# Autodesk Inventor assembly: Lightsaber Assembly 4
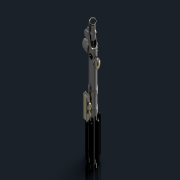
[picture p0: Inventor's stored thumbnail of the model, 180x180]
Saved by Autodesk Inventor 2021 (Build 250183000, 183)
## iProperties
Created: 2021-01-12
Part Number: Lightsaber Assembly 4
Document SubType Name: Assembly
Designer: Alex
Author: Alex
## Documents named in this file (13)
- D:\Documents (HDD)\lightsaber\Lightsaber Assembly 4.iam
- D:\Documents (HDD)\lightsaber\Grip.ipt
- D:\Documents (HDD)\lightsaber\Grip Base.ipt
- D:\Documents (HDD)\lightsaber\pin.ipt
- D:\Documents (HDD)\lightsaber\Middle handle.ipt
- D:\Documents (HDD)\lightsaber\top.ipt
- D:\Documents (HDD)\lightsaber\Clip.ipt
- D:\Documents (HDD)\lightsaber\Pin2.ipt
- D:\Documents (HDD)\lightsaber\Button1.ipt
- D:\Documents (HDD)\lightsaber\emitter.ipt
- D:\Documents (HDD)\lightsaber\Button.ipt
- D:\Documents (HDD)\lightsaber\Switch.ipt
- D:\Documents (HDD)\lightsaber\button 3.ipt
## Components (31 placed, 12 different names)
1. Grip:1 — Mate:1, Mate:2, Mate:49
2. Grip Base:1 — Mate:1, Mate:2, Mate:3, Mate:4, Mate:5, Mate:6, Mate:7, Mate:8, Mate:11, Mate:12, Mate:13, Mate:14, Insert:1, Insert:2, Insert:3, Insert:4, Insert:5, Insert:6, Insert:7, Insert:8, Insert:9, Insert:10, Insert:11, Insert:12, Mate:15, Mate:16, Mate:17
3. Grip:2 — Mate:3, Mate:4, Mate:45
4. Grip:3 — Mate:5, Mate:6, Mate:50
5. Grip:4 — Mate:7, Mate:8, Mate:48
6. Grip:5 — Mate:11, Mate:12, Mate:47
7. Grip:6 — Mate:13, Mate:14, Mate:46
8. pin:1 — Insert:10, Mate:46
9. pin:2 — Insert:9
10. pin:3 — Insert:11
11. pin:4 — Insert:12, Mate:50
12. pin:5 — Insert:7, Mate:47
13. pin:6 — Insert:8
14. pin:7 — Insert:5, Mate:48
15. pin:8 — Insert:6
16. pin:9 — Insert:2, Mate:49
17. pin:10 — Insert:4
18. pin:11 — Insert:1, Mate:45
19. pin:12 — Insert:3
20. Middle handle:1 — Mate:15, Mate:16, Mate:17, Mate:18, Mate:19, Mate:20, Mate:36, Mate:37, Mate:38, Angle:7, Flush:1
21. top:1 — Mate:18, Mate:19, Mate:20, Mate:22, Mate:23, Mate:24, Mate:25, Mate:26, Mate:27, Mate:28, Mate:29, Mate:30, Mate:31, Angle:1, Angle:2, Angle:3, Angle:4, Mate:32, Mate:33, Angle:5, Mate:34, Mate:35, Angle:6, Mate:42, Mate:43, Mate:44
22. Clip:1 — Mate:22, Mate:23
23. Pin2:1 — Mate:24, Mate:25, Angle:4
24. Pin2:2 — Mate:26, Mate:27, Angle:3
25. Pin2:3 — Mate:28, Mate:29, Angle:2
26. Pin2:4 — Mate:30, Mate:31, Angle:1
27. Button1:1 — Mate:32, Mate:33, Angle:5
28. emitter:1 — Mate:34, Mate:35, Angle:6
29. Button:1 — Mate:36, Mate:37, Mate:38, Angle:7, Flush:1, Angle:8, Mate:39, Mate:40, Mate:41
30. Switch:1 — Angle:8, Mate:39, Mate:40, Mate:41
31. button 3:1 — Mate:42, Mate:43, Mate:44
## Relationships (68: Mate 47, Insert 12, Angle 8, Flush 1)
- Mate:1: Grip:1 ↔ Grip Base:1
- Mate:2: Grip:1 ↔ Grip Base:1
- Mate:3: Grip Base:1 ↔ Grip:2
- Mate:4: Grip Base:1 ↔ Grip:2
- Mate:5: Grip Base:1 ↔ Grip:3
- Mate:6: Grip Base:1 ↔ Grip:3
- Mate:7: Grip Base:1 ↔ Grip:4
- Mate:8: Grip Base:1 ↔ Grip:4
- Mate:11: Grip Base:1 ↔ Grip:5
- Mate:12: Grip Base:1 ↔ Grip:5
- Mate:13: Grip Base:1 ↔ Grip:6
- Mate:14: Grip Base:1 ↔ Grip:6
- Insert:1: Grip Base:1 ↔ pin:11
- Insert:2: Grip Base:1 ↔ pin:9
- Insert:3: Grip Base:1 ↔ pin:12
- Insert:4: Grip Base:1 ↔ pin:10
- Insert:5: Grip Base:1 ↔ pin:7
- Insert:6: Grip Base:1 ↔ pin:8
- Insert:7: Grip Base:1 ↔ pin:5
- Insert:8: Grip Base:1 ↔ pin:6
- Insert:9: Grip Base:1 ↔ pin:2
- Insert:10: Grip Base:1 ↔ pin:1
- Insert:11: Grip Base:1 ↔ pin:3
- Insert:12: Grip Base:1 ↔ pin:4
- Mate:15: Grip Base:1 ↔ Middle handle:1
- Mate:16: Grip Base:1 ↔ Middle handle:1
- Mate:17: Grip Base:1 ↔ Middle handle:1
- Mate:18: Middle handle:1 ↔ top:1
- Mate:19: Middle handle:1 ↔ top:1
- Mate:20: Middle handle:1 ↔ top:1
- Mate:22: top:1 ↔ Clip:1
- Mate:23: top:1 ↔ Clip:1
- Mate:24: top:1 ↔ Pin2:1
- Mate:25: top:1 ↔ Pin2:1
- Mate:26: top:1 ↔ Pin2:2
- Mate:27: top:1 ↔ Pin2:2
- Mate:28: top:1 ↔ Pin2:3
- Mate:29: top:1 ↔ Pin2:3
- Mate:30: top:1 ↔ Pin2:4
- Mate:31: top:1 ↔ Pin2:4
- Angle:1 (180 deg): top:1 ↔ Pin2:4
- Angle:2 (0 deg): top:1 ↔ Pin2:3
- Angle:3 (0 deg): top:1 ↔ Pin2:2
- Angle:4 (0 deg): top:1 ↔ Pin2:1
- Mate:32: top:1 ↔ Button1:1
- Mate:33: top:1 ↔ Button1:1
- Angle:5 (0 deg): top:1 ↔ Button1:1
- Mate:34: top:1 ↔ emitter:1
- Mate:35: top:1 ↔ emitter:1
- Angle:6 (0 deg): top:1 ↔ emitter:1
- Mate:36: Middle handle:1 ↔ Button:1
- Mate:37: Middle handle:1 ↔ Button:1
- Mate:38: Middle handle:1 ↔ Button:1
- Angle:7 (0 deg): Middle handle:1 ↔ Button:1
- Flush:1: Middle handle:1 ↔ Button:1
- Angle:8 (0 deg): Button:1 ↔ Switch:1
- Mate:39: Button:1 ↔ Switch:1
- Mate:40 (1 mm): Button:1 ↔ Switch:1
- Mate:41 (1 mm): Button:1 ↔ Switch:1
- Mate:42: top:1 ↔ button 3:1
- Mate:43: top:1 ↔ button 3:1
- Mate:44: top:1 ↔ button 3:1
- Mate:45: Grip:2 ↔ pin:11
- Mate:46: Grip:6 ↔ pin:1
- Mate:47: Grip:5 ↔ pin:5
- Mate:48: Grip:4 ↔ pin:7
- Mate:49: Grip:1 ↔ pin:9
- Mate:50: Grip:3 ↔ pin:4
